# Autodesk Inventor assembly: XY Assembly
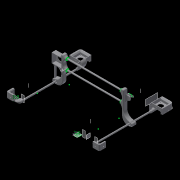
[picture p0: Inventor's stored thumbnail of the model, 180x180]
Saved by Autodesk Inventor 2014 (Build 180170000, 170)
## iProperties
Created: 2014-11-15
Part Number: XY Assembly
Document SubType Name: Assembly
Designer: Scott
Author: Scott
## Documents named in this file (8)
- C:\Users\Scott\Google Drive\Engineering Ideas and Designs\3D printer\Parts\XY Assembly.iam
- C:\Users\Scott\Google Drive\Engineering Ideas and Designs\3D printer\Parts\Ystart Right.ipt
- C:\Users\Scott\Google Drive\Engineering Ideas and Designs\3D printer\Parts\Bar.ipt
- C:\Users\Scott\Google Drive\Engineering Ideas and Designs\3D printer\Parts\Xcarriage Right.ipt
- C:\Users\Scott\Google Drive\Engineering Ideas and Designs\3D printer\Parts\Yend Right.ipt
- C:\Users\Scott\Google Drive\Engineering Ideas and Designs\3D printer\Parts\Xcarriage Left.ipt
- C:\Users\Scott\Google Drive\Engineering Ideas and Designs\3D printer\Parts\Ystart Left.ipt
- C:\Users\Scott\Google Drive\Engineering Ideas and Designs\3D printer\Parts\Yend Left.ipt
## Components (10 placed, 7 different names)
1. Ystart Right:1 — Insert:1
2. Bar:1 — Insert:1, Insert:2, Mate:1, Insert:3
3. Xcarriage Right:1 — Insert:2, Mate:2, Insert:4, Insert:5
4. Yend Right:1 — Mate:1, Insert:3
5. Bar:2 — Insert:5, Insert:8
6. Bar:3 — Mate:2, Insert:4, Insert:7
7. Xcarriage Left:1 — Insert:7, Insert:8, Insert:9
8. Bar:4 — Insert:9, Insert:10, Insert:11
9. Ystart Left:1 — Insert:10
10. Yend Left:1 — Insert:11
## Relationships (12: Insert 10, Mate 2)
- Insert:1: Ystart Right:1 ↔ Bar:1
- Insert:2 (-203.2 mm): Bar:1 ↔ Xcarriage Right:1
- Mate:1: Bar:1 ↔ Yend Right:1
- Insert:3: Bar:1 ↔ Yend Right:1
- Mate:2: Xcarriage Right:1 ↔ Bar:3
- Insert:4: Xcarriage Right:1 ↔ Bar:3
- Insert:5: Xcarriage Right:1 ↔ Bar:2
- Insert:7: Bar:3 ↔ Xcarriage Left:1
- Insert:8: Bar:2 ↔ Xcarriage Left:1
- Insert:9 (-121.92 mm): Xcarriage Left:1 ↔ Bar:4
- Insert:10: Bar:4 ↔ Ystart Left:1
- Insert:11: Bar:4 ↔ Yend Left:1
